# Autodesk Inventor assembly: Control_1
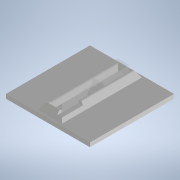
[picture p0: Inventor's stored thumbnail of the model, 180x180]
Saved by Autodesk Inventor 2021 (Build 250183000, 183)
## iProperties
Created: 2022-02-21
Part Number: Control_1
Document SubType Name: Assembly
Designer: aerts
Author: aerts
## Documents named in this file (3)
- C:\Users\aerts\Desktop\Project\3D\Control_1.iam
- C:\Users\aerts\Desktop\Project\3D\Weight_Sensor.ipt
- C:\Users\aerts\Desktop\Project\3D\Weight_Plate.ipt
## Components (2 placed, 2 different names)
1. Weight_Sensor:1 — Mate:1, Mate:2, Mate:3
2. Weight_Plate:1 — Mate:1, Mate:2, Mate:3
## Relationships (3: Mate 3)
- Mate:1: Weight_Sensor:1 ↔ Weight_Plate:1
- Mate:2: Weight_Sensor:1 ↔ Weight_Plate:1
- Mate:3: Weight_Sensor:1 ↔ Weight_Plate:1
